# Autodesk Inventor assembly: entireRobot
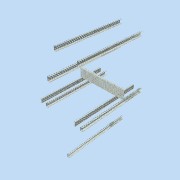
[picture p0: Inventor's stored thumbnail of the model, 180x180]
Saved by Autodesk Inventor 2015 (Build 190159000, 159)
## iProperties
Created: 2017-06-02
Part Number: entireRobot
Document SubType Name: Assembly
Designer: Tommy
Author: Tommy
## Documents named in this file (3)
- C:\Users\Tommy\Documents\GitHub\VEX-Robotics-2017-2018\Robot\entireRobot.iam
- C:\Users\Tommy\Documents\GitHub\VEX-Robotics-2017-2018\Imperial\Structure\C-Channel 1x5x1x35 Hole.iam
- C:\Users\Tommy\Documents\GitHub\VEX-Robotics-2017-2018\Imperial\Structure\C-Channel 1x5x1x25 Hole.ipt
## Components (9 placed, 2 different names)
1. C-Channel 1x5x1x35 Hole:1 [sub-assembly] — Mate:1, Flush:1, Flush:2, Flush:3
2. C-Channel 1x5x1x35 Hole:2 [sub-assembly] — Mate:2, Flush:2, Flush:5, Flush:8
3. C-Channel 1x5x1x35 Hole:3 [sub-assembly]
4. C-Channel 1x5x1x35 Hole:4 [sub-assembly]
5. C-Channel 1x5x1x35 Hole:5 [sub-assembly]
6. C-Channel 1x5x1x35 Hole:6 [sub-assembly] — Mate:5, Flush:6, Flush:7
7. C-Channel 1x5x1x35 Hole:7 [sub-assembly] — Mate:4, Flush:4, Flush:5, Flush:6
8. C-Channel 1x5x1x35 Hole:8 [sub-assembly]
9. C-Channel 1x5x1x25 Hole:1 — Mate:1, Flush:1, Mate:2, Flush:3, Mate:4, Flush:4, Mate:5, Flush:7, Flush:8
## Relationships (12: Flush 8, Mate 4)
- Mate:1: C-Channel 1x5x1x35 Hole:1 ↔ C-Channel 1x5x1x25 Hole:1
- Flush:1: C-Channel 1x5x1x35 Hole:1 ↔ C-Channel 1x5x1x25 Hole:1
- Mate:2: C-Channel 1x5x1x35 Hole:2 ↔ C-Channel 1x5x1x25 Hole:1
- Flush:2: C-Channel 1x5x1x35 Hole:1 ↔ C-Channel 1x5x1x35 Hole:2
- Flush:3: C-Channel 1x5x1x35 Hole:1 ↔ C-Channel 1x5x1x25 Hole:1
- Mate:4: C-Channel 1x5x1x35 Hole:7 ↔ C-Channel 1x5x1x25 Hole:1
- Flush:4: C-Channel 1x5x1x35 Hole:7 ↔ C-Channel 1x5x1x25 Hole:1
- Flush:5: C-Channel 1x5x1x35 Hole:2 ↔ C-Channel 1x5x1x35 Hole:7
- Mate:5: C-Channel 1x5x1x35 Hole:6 ↔ C-Channel 1x5x1x25 Hole:1
- Flush:6: C-Channel 1x5x1x35 Hole:6 ↔ C-Channel 1x5x1x35 Hole:7
- Flush:7: C-Channel 1x5x1x35 Hole:6 ↔ C-Channel 1x5x1x25 Hole:1
- Flush:8: C-Channel 1x5x1x35 Hole:2 ↔ C-Channel 1x5x1x25 Hole:1
